# Autodesk Inventor assembly: !structure
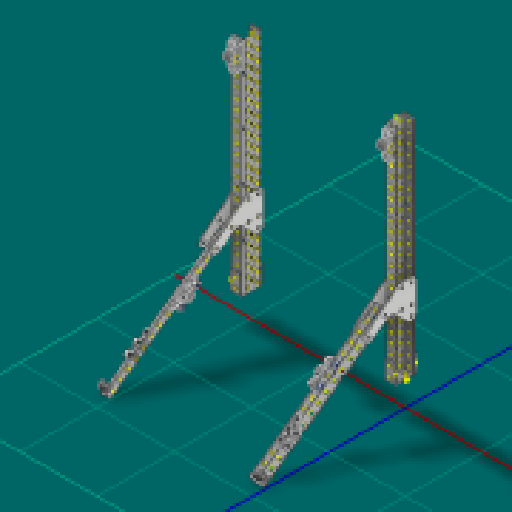
[picture p0: Inventor's stored thumbnail of the model, 512x512]
Saved by Autodesk Inventor 2025 (Build 290162000, 162)
## iProperties
Created: 2024-10-13
Part Number: !structure
Document SubType Name: Assembly
Designer: Averey Ku
Author: Averey Ku
## Documents named in this file (3)
- C:\Users\avere\vex_robotics_high_stakes\hardware\cad\bots\high_stakes_v2\tower\structure\!structure.iam
- C:\Users\avere\vex_robotics_high_stakes\hardware\cad\bots\high_stakes_v2\tower\structure\side.iam
- C:\Users\avere\vex_robotics_high_stakes\hardware\cad\bots\high_stakes_v2\tower\structure\side_mirrored\side_mirrored.iam
## Components (2 placed, 2 different names)
1. side:1 [sub-assembly] — Mate:2
2. side_mirrored:1 [sub-assembly]
## Relationships (3: Mate 2, Insert 1)
- [Insert] (187.325 mm): side:1 ↔ side_mirrored:1
- [Mate]: side:1 ↔ side_mirrored:1
- Mate:2: side:1
